# Autodesk Inventor assembly: Chassis
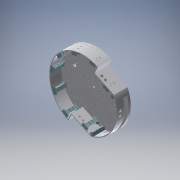
[picture p0: Inventor's stored thumbnail of the model, 180x180]
Saved by Autodesk Inventor 2017 SP1 (Build 210196100, 196)
## iProperties
Created: 2017-05-15
Part Number: Chassis
Document SubType Name: Assembly
Designer: zallen
Mass: 2683.15 g
Surface Area: 5804.94 cm^2
Volume: 2531.27 cm^3
Density: 1.06 g/cm^3
Author: zallen
## Documents named in this file (15)
- C:\Users\Zach\Documents\Autodesk Inventor Projects\LaundryRobot_v0.1\Base\Chassis - Modular\Chassis.iam
- C:\Users\Zach\Documents\Autodesk Inventor Projects\LaundryRobot_v0.1\Base\Chassis - Modular\SB075.ipt
- C:\Users\Zach\Documents\Autodesk Inventor Projects\LaundryRobot_v0.1\Base\Chassis - Modular\CP001.ipt
- C:\Users\Zach\Documents\Autodesk Inventor Projects\LaundryRobot_v0.1\Base\Chassis - Modular\CP002.ipt
- C:\Users\Zach\Documents\Autodesk Inventor Projects\LaundryRobot_v0.1\Base\Chassis - Modular\CP003.ipt
- C:\Users\Zach\Documents\Autodesk Inventor Projects\LaundryRobot_v0.1\Base\Chassis - Modular\CP004.ipt
- C:\Users\Zach\Documents\Autodesk Inventor Projects\LaundryRobot_v0.1\Base\Chassis - Modular\CP005.ipt
- C:\Users\Zach\Documents\Autodesk Inventor Projects\LaundryRobot_v0.1\Base\Chassis - Modular\CP006.ipt
- C:\Users\Zach\Documents\Autodesk Inventor Projects\LaundryRobot_v0.1\Base\Chassis - Modular\CP007.ipt
- C:\Users\Zach\Documents\Autodesk Inventor Projects\LaundryRobot_v0.1\Base\Chassis - Modular\CP008.ipt
- C:\Users\Zach\Documents\Autodesk Inventor Projects\LaundryRobot_v0.1\Base\Chassis - Modular\CP009.ipt
- C:\Users\Zach\Documents\Autodesk Inventor Projects\LaundryRobot_v0.1\Base\Chassis - Modular\CP010.ipt
- C:\Users\Zach\Documents\Autodesk Inventor Projects\LaundryRobot_v0.1\Base\Chassis - Modular\CP011.ipt
- C:\Users\Zach\Documents\Autodesk Inventor Projects\LaundryRobot_v0.1\Base\Chassis - Modular\CP012.ipt
- C:\Users\Zach\Documents\Autodesk Inventor Projects\LaundryRobot_v0.1\Base\Chassis - Modular\CW000.ipt
## Components (33 placed, 14 different names)
1. SB075:1 — Mate:3, Mate:5, Mate:118, Mate:121, Flush:1
2. SB075:2 — Mate:3, Mate:5, Mate:120
3. CP002:1 — Mate:9, Mate:10, Mate:80, Mate:81, Mate:82, Mate:115, Mate:117, Mate:119, Mate:136
4. CP003:1 — Mate:9, Mate:10, Mate:99, Mate:101, Mate:132, Mate:134
5. CP004:1 — Mate:98, Mate:99, Mate:101, Mate:109, Mate:126, Mate:128, Mate:137
6. CP001:2 — Mate:23, Mate:24, Mate:35, Mate:36, Mate:37, Mate:55, Mate:102, Mate:105, Mate:106
7. CP005:1 — Mate:23, Mate:24, Mate:25, Mate:26, Mate:27, Mate:40, Mate:41, Mate:42, Mate:53, Mate:62, Mate:103
8. CP006:1 — Mate:25, Mate:26, Mate:27, Mate:30, Mate:31, Mate:32, Mate:46, Mate:48, Mate:58
9. SB075:3 — Mate:30, Flush:3
10. SB075:4 — Mate:31, Mate:32
11. SB075:5 — Mate:35, Mate:37
12. SB075:6 — Mate:36, Flush:6
13. SB075:7 — Mate:40, Flush:4
14. SB075:8 — Mate:41, Mate:42
15. SB075:9 — Mate:46, Mate:47, Mate:48
16. SB075:10 — Mate:47, Flush:2
17. SB075:11 — Mate:55
18. SB075:12 — Mate:53, Flush:5
19. CP007:1 — Mate:58, Mate:60, Mate:66, Mate:67, Mate:68, Mate:70, Mate:75, Mate:77, Mate:113, Mate:114, Mate:116
20. CP007:2 — Mate:60, Mate:62, Mate:63, Mate:65, Mate:73, Mate:74, Mate:102, Mate:103
21. CP008:1 — Mate:63, Mate:65, Mate:72, Mate:98, Mate:107, Mate:112
22. CP009:1 — Mate:66, Mate:67, Mate:68, Mate:71, Mate:119, Flush:9
23. CP010:1 — Mate:70, Mate:71, Mate:72
24. CP010:2 — Mate:73, Mate:74, Mate:75, Mate:77
25. SB075:13 — Mate:80, Mate:82
26. SB075:14 — Mate:81
27. SB075:15 — Mate:108, Mate:110
28. SB075:16 — Mate:111
29. CP011:1 — Mate:105, Mate:106, Mate:107, Mate:108, Mate:109, Mate:110, Mate:111, Mate:112
30. CP012:1 — Mate:113, Mate:114, Mate:115, Mate:116, Mate:117, Mate:118, Mate:120, Mate:121
31. SB075:17 — Mate:126, Mate:128, Flush:7
32. SB075:19 — Mate:132, Mate:134, Flush:8
33. CW000:1 — Mate:136, Mate:137, Flush:1, Flush:2, Flush:3, Flush:4, Flush:5, Flush:6, Flush:7, Flush:8
## Relationships (93: Mate 84, Flush 9)
- Mate:3: SB075:1 ↔ SB075:2
- Mate:5: SB075:1 ↔ SB075:2
- Mate:9: CP002:1 ↔ CP003:1
- Mate:10: CP002:1 ↔ CP003:1
- Mate:23: CP001:2 ↔ CP005:1
- Mate:24: CP001:2 ↔ CP005:1
- Mate:25: CP005:1 ↔ CP006:1
- Mate:26: CP005:1 ↔ CP006:1
- Mate:27: CP005:1 ↔ CP006:1
- [Mate]: SB075:3 ↔ SB075:4
- [Mate]: SB075:3 ↔ SB075:4
- Mate:30: CP006:1 ↔ SB075:3
- Mate:31: CP006:1 ↔ SB075:4
- Mate:32: CP006:1 ↔ SB075:4
- [Mate]: SB075:5 ↔ SB075:6
- [Mate]: SB075:5 ↔ SB075:6
- Mate:35: CP001:2 ↔ SB075:5
- Mate:36: CP001:2 ↔ SB075:6
- Mate:37: CP001:2 ↔ SB075:5
- [Mate]: SB075:7 ↔ SB075:8
- [Mate]: SB075:7 ↔ SB075:8
- Mate:40: CP005:1 ↔ SB075:7
- Mate:41: CP005:1 ↔ SB075:8
- Mate:42: CP005:1 ↔ SB075:8
- [Mate]: SB075:9 ↔ SB075:10
- [Mate]: SB075:9 ↔ SB075:10
- Mate:46: CP006:1 ↔ SB075:9
- Mate:47: SB075:9 ↔ SB075:10
- Mate:48: CP006:1 ↔ SB075:9
- [Mate]: SB075:11 ↔ SB075:12
- [Mate]: SB075:11 ↔ SB075:12
- [Mate]: SB075:11 ↔ SB075:12
- Mate:53: CP005:1 ↔ SB075:12
- Mate:55: CP001:2 ↔ SB075:11
- Mate:58: CP006:1 ↔ CP007:1
- Mate:60: CP007:1 ↔ CP007:2
- Mate:62: CP005:1 ↔ CP007:2
- Mate:63: CP007:2 ↔ CP008:1
- Mate:65: CP007:2 ↔ CP008:1
- Mate:66: CP007:1 ↔ CP009:1
- Mate:67: CP007:1 ↔ CP009:1
- Mate:68: CP007:1 ↔ CP009:1
- Mate:70: CP007:1 ↔ CP010:1
- Mate:71: CP009:1 ↔ CP010:1
- Mate:72: CP008:1 ↔ CP010:1
- Mate:73: CP007:2 ↔ CP010:2
- Mate:74: CP007:2 ↔ CP010:2
- Mate:75: CP007:1 ↔ CP010:2
- Mate:77: CP007:1 ↔ CP010:2
- [Mate]: SB075:13 ↔ SB075:14
- [Mate]: SB075:13 ↔ SB075:14
- Mate:80: CP002:1 ↔ SB075:13
- Mate:81: CP002:1 ↔ SB075:14
- Mate:82: CP002:1 ↔ SB075:13
- [Mate]: SB075:15 ↔ SB075:16
- [Mate]: SB075:15 ↔ SB075:16
- Mate:98: CP004:1 ↔ CP008:1
- Mate:99: CP003:1 ↔ CP004:1
- Mate:101: CP003:1 ↔ CP004:1
- Mate:102: CP001:2 ↔ CP007:2
- Mate:103: CP005:1 ↔ CP007:2
- Mate:105: CP001:2 ↔ CP011:1
- Mate:106: CP001:2 ↔ CP011:1
- Mate:107: CP008:1 ↔ CP011:1
- Mate:108: SB075:15 ↔ CP011:1
- Mate:109: CP004:1 ↔ CP011:1
- Mate:110: SB075:15 ↔ CP011:1
- Mate:111: SB075:16 ↔ CP011:1
- Mate:112: CP008:1 ↔ CP011:1
- Mate:113: CP007:1 ↔ CP012:1
- Mate:114: CP007:1 ↔ CP012:1
- Mate:115: CP002:1 ↔ CP012:1
- Mate:116: CP007:1 ↔ CP012:1
- Mate:117: CP002:1 ↔ CP012:1
- Mate:118: SB075:1 ↔ CP012:1
- Mate:119: CP002:1 ↔ CP009:1
- Mate:120: SB075:2 ↔ CP012:1
- Mate:121: SB075:1 ↔ CP012:1
- Mate:126: CP004:1 ↔ SB075:17
- Mate:128: CP004:1 ↔ SB075:17
- Mate:132: CP003:1 ↔ SB075:19
- Mate:134: CP003:1 ↔ SB075:19
- Mate:136: CP002:1 ↔ CW000:1
- Mate:137: CP004:1 ↔ CW000:1
- Flush:1: SB075:1 ↔ CW000:1
- Flush:2: SB075:10 ↔ CW000:1
- Flush:3: SB075:3 ↔ CW000:1
- Flush:4: SB075:7 ↔ CW000:1
- Flush:5: SB075:12 ↔ CW000:1
- Flush:6: SB075:6 ↔ CW000:1
- Flush:7: SB075:17 ↔ CW000:1
- Flush:8: SB075:19 ↔ CW000:1
- Flush:9: CP009:1
## Named parameters: d32_d4 = 0 mm, d33_d2 = 0 mm, d37_d32_d4 = 0 mm, d38_d33_d2 = 0 mm, d42_d37_d32_d4 = 0 mm, d43_d38_d33_d2 = 0 mm, d47_d42_d37_d32_d4 = 0 mm, d48_d43_d38_d33_d2 = 0 mm, d54_d51 = 0 mm, d55_d47_d42_d37_d32_d4 = 0 mm, d56_d48_d43_d38_d33_d2 = 0 mm, d90_d2 = 0 mm, d91_d4 = 0 mm, d101_d2 = 0 mm, d102_d4 = 0 mm
